# Autodesk Inventor assembly: Pickup Motor
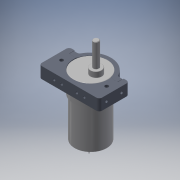
[picture p0: Inventor's stored thumbnail of the model, 180x180]
Saved by Autodesk Inventor 2016 (Build 200138000, 138)
## iProperties
Created: 2015-11-25
Part Number: Pickup Motor
Document SubType Name: Assembly
Designer: Julia
Author: Julia
## Documents named in this file (4)
- C:\Users\Julia\Documents\GitHub\RobotuxCAD\FTC CAD Parts\Pickup Motor.iam
- C:\Users\Julia\Documents\GitHub\RobotuxCAD\FTC CAD Parts\FTC 2015 - 2016 Season Solidworks\Solidworks_Team\FTC KOP 2015 - 2016\Tetrix Elements\Tetrix_Parts\Motors\Full motor model.ipt
- C:\Users\Julia\Documents\GitHub\RobotuxCAD\FTC CAD Parts\Tetrix_Kit_FTC\tetrix_739376x108129_2013.ipt
- C:\Users\Julia\Documents\GitHub\RobotuxCAD\FTC CAD Parts\Tetrix_Kit_FTC\tetrix_739376x108128_2013.ipt
## Components (3 placed, 3 different names)
1. Full motor model:1 — Mate:1, Flush:1
2. tetrix_739376x108129_2013:1 — Mate:1, Mate:2, Mate:3, Mate:4, Flush:1
3. tetrix_739376x108128_2013:1 — Mate:2, Mate:3, Mate:4
## Relationships (5: Mate 4, Flush 1)
- Mate:1: Full motor model:1 ↔ tetrix_739376x108129_2013:1
- Mate:2: tetrix_739376x108129_2013:1 ↔ tetrix_739376x108128_2013:1
- Mate:3: tetrix_739376x108129_2013:1 ↔ tetrix_739376x108128_2013:1
- Mate:4: tetrix_739376x108129_2013:1 ↔ tetrix_739376x108128_2013:1
- Flush:1: Full motor model:1 ↔ tetrix_739376x108129_2013:1
